# Autodesk Inventor assembly: Sub.Rueda
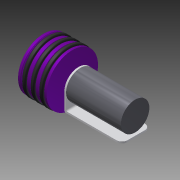
[picture p0: Inventor's stored thumbnail of the model, 180x180]
Saved by Autodesk Inventor 2014 (Build 180170000, 170)
## iProperties
Created: 2014-01-26
Part Number: Sub.Rueda
Document SubType Name: Assembly
Designer: Sanjo
Mass: 111.528 g
Surface Area: 219.129 cm^2
Volume: 63.3799 cm^3
Density: 1.75967 g/cm^3
Author: Sanjo
## Documents named in this file (7)
- C:\Users\Rubén\Desktop\Robot Sumo\Piezas\Sub.Rueda.iam
- C:\Users\Rubén\Desktop\Robot Sumo\Piezas\Brida Sujección Motor.ipt
- C:\Users\Rubén\Desktop\Robot Sumo\Piezas\Motor.ipt
- C:\Users\Rubén\Desktop\Robot Sumo\Piezas\Rueda.ipt
- C:\Users\Rubén\Desktop\Robot Sumo\Piezas\Tornillo M3x5.ipt
- C:\Users\Rubén\Desktop\Robot Sumo\Piezas\Sub.Rueda\Design Accelerator\Junta tórica1.iam
- C:\Users\Rubén\Desktop\Robot Sumo\Piezas\Sub.Rueda\Design Accelerator\Conexión de pasador radial1.iam
## Components (9 placed, 6 different names)
1. Brida Sujección Motor:1 — Insertar:1, Insertar:2, Insertar:3, Insertar:4, Insertar:5, Insertar:6, Coincidencia:2
2. Motor:1 — Insertar:5, Insertar:6, Coincidencia:1
3. Rueda:1 — Coincidencia:1, Coincidencia:2, Coincidencia:3, Coincidencia:4, Coincidencia:5, Coincidencia:6
4. Tornillo M3x5:1 — Insertar:4
5. Tornillo M3x5:2 — Insertar:2
6. Tornillo M3x5:3 — Insertar:3
7. Tornillo M3x5:4 — Insertar:1
8. Junta tórica:1 [sub-assembly] — Coincidencia:3, Coincidencia:4
9. Conexión de pasador radial:1 [sub-assembly] — Coincidencia:5, Coincidencia:6
## Relationships (12: Insert 6, Mate 6)
- Insertar:1: Brida Sujección Motor:1 ↔ Tornillo M3x5:4
- Insertar:2: Brida Sujección Motor:1 ↔ Tornillo M3x5:2
- Insertar:3: Brida Sujección Motor:1 ↔ Tornillo M3x5:3
- Insertar:4: Brida Sujección Motor:1 ↔ Tornillo M3x5:1
- Insertar:5: Brida Sujección Motor:1 ↔ Motor:1
- Insertar:6: Brida Sujección Motor:1 ↔ Motor:1
- Coincidencia:1 [Mate]: Motor:1 ↔ Rueda:1
- Coincidencia:2 [Mate] (0.5 mm): Brida Sujección Motor:1 ↔ Rueda:1
- Coincidencia:3 [Mate]: Rueda:1 ↔ Junta tórica:1
- Coincidencia:4 [Mate]: Rueda:1 ↔ Junta tórica:1
- Coincidencia:5 [Mate]: Rueda:1 ↔ Conexión de pasador radial:1
- Coincidencia:6 [Mate]: Rueda:1 ↔ Conexión de pasador radial:1
